# Autodesk Inventor assembly: Übertragung des Zahnriemens
Saved by Autodesk Inventor 2016 (Build 200138000, 138)
## iProperties
Created: 2015-08-24
Part Number: Übertragung des Zahnriemens
Document SubType Name: Assembly
Designer: 4ndreas
ClientObjectVersion: 1
Author: 4ndreas
## Documents named in this file (8)
- C:\Users\4ndreas\Documents\Inventor\RobotARM v2\v4\Ellbow\Konstruktions-Assistent\Übertragung des Zahnriemens1.iam
- C:\Users\4ndreas\Documents\Inventor\RobotARM v2\v4\Ellbow\Konstruktions-Assistent\Zahnriemen1.ipt
- C:\Users\4ndreas\Documents\Inventor\RobotARM v2\v4\Ellbow\Konstruktions-Assistent\Synchrone Riemenscheibe11.ipt
- C:\Users\4ndreas\Documents\Inventor\RobotARM v2\v4\Ellbow\Konstruktions-Assistent\Flache Riemenscheibe21.ipt
- C:\Users\4ndreas\Documents\Inventor\RobotARM v2\v4\Ellbow\Konstruktions-Assistent\Synchrone Riemenscheibe21.ipt
- C:\Users\4ndreas\Documents\Inventor\RobotARM v2\v4\Ellbow\Konstruktions-Assistent\Flache Riemenscheibe11.ipt
- C:\Users\4ndreas\Documents\Inventor\RobotARM v2\v4\Ellbow\Konstruktions-Assistent\Flache Riemenscheibe41.ipt
- C:\Users\4ndreas\Documents\Inventor\RobotARM v2\v4\Ellbow\Konstruktions-Assistent\Flache Riemenscheibe31.ipt
## Components (7 placed, 7 different names)
1. Zahnriemen:1 — Fluchtend:1, Passend:1, Passend:2, Fluchtend:2, Passend:3, Fluchtend:3, Passend:4, Fluchtend:4, Passend:5, Passend:6, Fluchtend:5, Passend:7, Fluchtend:6, Passend:8
2. Synchrone Riemenscheibe1:1 — Fluchtend:1, Passend:1, Passend:2, Drehung:1, Drehung:2, Drehung:3, Drehung:4, Drehung:5
3. Flache Riemenscheibe2:1 — Fluchtend:3, Passend:4, Drehung:2
4. Synchrone Riemenscheibe2:1 — Fluchtend:4, Passend:5, Drehung:3, Passend:6
5. Flache Riemenscheibe1:1 — Fluchtend:5, Passend:7, Drehung:4
6. Flache Riemenscheibe4:1 — Fluchtend:2, Passend:3, Drehung:1
7. Flache Riemenscheibe3:1 — Fluchtend:6, Passend:8, Drehung:5
## Relationships (19: Mate 8, Flush 6, RelateRotation 5)
- Fluchtend:1 [Flush]: Zahnriemen:1 ↔ Synchrone Riemenscheibe1:1
- Passend:1 [Mate]: Zahnriemen:1 ↔ Synchrone Riemenscheibe1:1
- Passend:2 [Mate]: Zahnriemen:1 ↔ Synchrone Riemenscheibe1:1
- Fluchtend:2 [Flush]: Zahnriemen:1 ↔ Flache Riemenscheibe4:1
- Passend:3 [Mate]: Zahnriemen:1 ↔ Flache Riemenscheibe4:1
- Drehung:1 [RelateRotation] (0.1466 ul): Synchrone Riemenscheibe1:1 ↔ Flache Riemenscheibe4:1
- Fluchtend:3 [Flush]: Zahnriemen:1 ↔ Flache Riemenscheibe2:1
- Passend:4 [Mate]: Zahnriemen:1 ↔ Flache Riemenscheibe2:1
- Drehung:2 [RelateRotation] (0.1466 ul): Synchrone Riemenscheibe1:1 ↔ Flache Riemenscheibe2:1
- Fluchtend:4 [Flush]: Zahnriemen:1 ↔ Synchrone Riemenscheibe2:1
- Passend:5 [Mate]: Zahnriemen:1 ↔ Synchrone Riemenscheibe2:1
- Drehung:3 [RelateRotation] (0.2667 ul): Synchrone Riemenscheibe1:1 ↔ Synchrone Riemenscheibe2:1
- Passend:6 [Mate]: Zahnriemen:1 ↔ Synchrone Riemenscheibe2:1
- Fluchtend:5 [Flush]: Zahnriemen:1 ↔ Flache Riemenscheibe1:1
- Passend:7 [Mate]: Zahnriemen:1 ↔ Flache Riemenscheibe1:1
- Drehung:4 [RelateRotation] (0.1466 ul): Synchrone Riemenscheibe1:1 ↔ Flache Riemenscheibe1:1
- Fluchtend:6 [Flush]: Zahnriemen:1 ↔ Flache Riemenscheibe3:1
- Passend:8 [Mate]: Zahnriemen:1 ↔ Flache Riemenscheibe3:1
- Drehung:5 [RelateRotation] (0.1466 ul): Synchrone Riemenscheibe1:1 ↔ Flache Riemenscheibe3:1
